# Autodesk Inventor assembly: motor_module
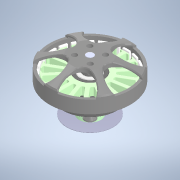
[picture p0: Inventor's stored thumbnail of the model, 180x180]
Saved by Autodesk Inventor 2022.2 (Build 262287000, 287)
## iProperties
Created: 2016-08-15
Part Number: motor_module
Document SubType Name: Assembly
Designer: Jochen
Sending System: SolidWorks 2017
Last Author: Felix
Last Saved: 2021-02-23
Author: Jochen
## Documents named in this file (7)
- D:\Projects\Lisbeth\CAD\Common\Motor\MotorModule.iam
- D:\Projects\Lisbeth\CAD\Common\Motor\motor_antigravity_4004_custom_shaft.iam
- D:\Projects\Lisbeth\CAD\Common\Encoder\EncoderCodeWheelMount.ipt
- D:\Projects\Lisbeth\CAD\Common\Encoder\encoder_codewheel_5000cpr_pwb_7mm.ipt
- D:\Projects\Lisbeth\CAD\Common\Motor\bearing_8_4_2_sbn_MR84VA.ipt
- D:\Projects\Lisbeth\CAD\Common\Motor\fastener_fhs_m3_5.ipt
- D:\Projects\Lisbeth\CAD\Common\Motor\TransmissionPulleyMotor.ipt
## Components (9 placed, 6 different names)
1. motor_antigravity_4004_custom_shaft:2 [sub-assembly] — Mate:6, Mate:7, Mate:8, Mate:11
2. encoder_codewheel_pwb_mount:1 — Mate:8, Mate:9, Mate:10, Mate:12, Mate:13
3. encoder_codewheel_5000cpr_pwb_7mm:1 — Mate:10, Mate:13
4. bearing_8_4_2_sbn_MR84VA:1 — Mate:6, Mate:7, Mate:9
5. fastener_fhs_m3_5:3
6. fastener_fhs_m3_5:1
7. fastener_fhs_m3_5:4
8. fastener_fhs_m3_5:2
9. TransmissionPulleyMotor:1 — Mate:11, Mate:12
## Relationships (8: Mate 8)
- Mate:6: motor_antigravity_4004_custom_shaft:2 ↔ bearing_8_4_2_sbn_MR84VA:1
- Mate:7: motor_antigravity_4004_custom_shaft:2 ↔ bearing_8_4_2_sbn_MR84VA:1
- Mate:8: motor_antigravity_4004_custom_shaft:2 ↔ encoder_codewheel_pwb_mount:1
- Mate:9: encoder_codewheel_pwb_mount:1 ↔ bearing_8_4_2_sbn_MR84VA:1
- Mate:10: encoder_codewheel_pwb_mount:1 ↔ encoder_codewheel_5000cpr_pwb_7mm:1
- Mate:11: motor_antigravity_4004_custom_shaft:2 ↔ TransmissionPulleyMotor:1
- Mate:12: encoder_codewheel_pwb_mount:1 ↔ TransmissionPulleyMotor:1
- Mate:13: encoder_codewheel_pwb_mount:1 ↔ encoder_codewheel_5000cpr_pwb_7mm:1
